# Autodesk Inventor assembly: Assembly1
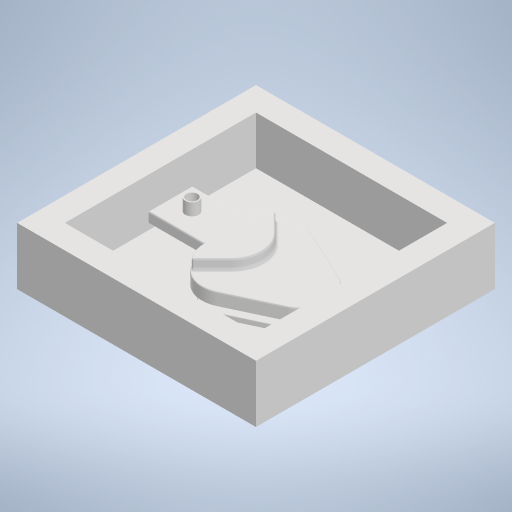
[picture p0: Inventor's stored thumbnail of the model, 512x512]
Saved by Autodesk Inventor 2024.3 (Build 283343000, 343)
## iProperties
Created: 2025-06-26
Part Number: Assembly1
Document SubType Name: Assembly
Designer: 1
Author: 1
## Documents named in this file (3)
- F:\UMN Researches\CUHK Research\SKIN\Assembly1.iam
- F:\UMN Researches\CUHK Research\SKIN\Box.ipt
- F:\UMN Researches\CUHK Research\SKIN\Product Model.ipt
## Components (2 placed, 2 different names)
1. Box:1 — Mate:1, Mate:2, Mate:3, Flush:1
2. Product Model:1 — Mate:1, Mate:2, Mate:3, Flush:1
## Relationships (4: Mate 3, Flush 1)
- Mate:1: Box:1 ↔ Product Model:1
- Mate:2 (20 mm): Box:1 ↔ Product Model:1
- Mate:3 (66.7 mm): Box:1 ↔ Product Model:1
- Flush:1: Box:1 ↔ Product Model:1
